# Autodesk Inventor assembly: Project Integration copy
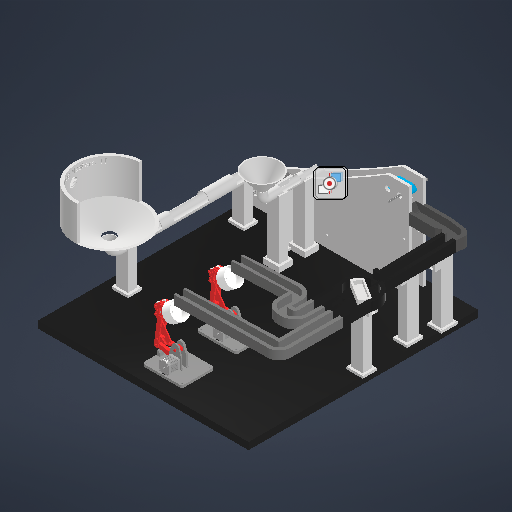
[picture p0: Inventor's stored thumbnail of the model, 512x512]
Saved by Autodesk Inventor 2025.2 (Build 292293000, 293)
## iProperties
Created: 2026-04-17
Part Number: Project Integration copy
Document SubType Name: Assembly
Designer: manon
Author: manon
## Documents named in this file (19)
- C:\Users\osama\Downloads\Project Integration copy .iam
- C:\Users\osama\Downloads\base.ipt
- C:\Users\osama\Downloads\Sorting Path.ipt
- C:\Users\osama\Downloads\Sorting Gate Edited (1).ipt
- C:\Users\osama\Downloads\Assembly Micro Servo MG90S (2) (1).iam
- C:\Users\osama\Downloads\SG90 Horn.ipt
- C:\Users\osama\Downloads\lifting assembly.iam
- C:\Users\osama\Downloads\Path to Sorting Final.ipt
- C:\Users\osama\Downloads\Left Path Final.ipt
- C:\Users\osama\Downloads\Right Path Final.ipt
- C:\Users\osama\Downloads\select support through rabie.ipt
- C:\Users\osama\Downloads\hoop.ipt
- C:\Users\osama\Downloads\support of collector.ipt
- C:\Users\osama\Downloads\path to lifting.ipt
- C:\Users\osama\Downloads\mg996R_v2.ipt
- C:\Users\osama\Downloads\starting point.ipt
- C:\Users\osama\Downloads\Full Assembly.ipt
- C:\Users\osama\Downloads\support of collector copy.ipt
- C:\Users\osama\Downloads\scoop.ipt
## Components (25 placed, 18 different names)
1. base:2 — Mate:26, Mate:27, Mate:57, Mate:58, Mate:62, Mate:68, Mate:72, Mate:76, Mate:88, Mate:89, Mate:96, Mate:99, Mate:100, Mate:101
2. Sorting Path:1 — Mate:5, Mate:6, Mate:43, Mate:44, Mate:45, Mate:46, Mate:47, Mate:48, Mate:50, Mate:55, Mate:90, Mate:91
3. Sorting Gate Edited (1):1 — Mate:5, Mate:6, Rigid:1
4. Assembly Micro Servo MG90S (2) (1):1 [sub-assembly] — Mate:7, Mate:8
5. SG90 Horn:2 — Mate:7, Mate:8, Rigid:1
6. lifting assembly:1 [sub-assembly] — Mate:26, Mate:27, Mate:28, Mate:29, Mate:31
7. Path to Sorting Final:1 — Mate:28, Mate:29, Mate:31
8. Left Path Final:1 — Mate:46, Mate:47, Mate:48
9. Right Path Final:1 — Mate:43, Mate:44, Mate:45
10. select support through rabie:1 — Mate:50, Mate:90
11. select support through rabie:2 — Mate:89, Mate:91
12. select support through rabie:3 — Mate:55, Mate:88
13. hoop:1
14. support of collector:1 — Mate:58, Mate:62
15. support of collector:2 — Mate:57
16. path to lifting:1
17. mg996R_v2:1 — Mate:73, Mate:74, Mate:75, Mate:77, Mate:78, Mate:87
18. starting point:1 — Mate:79, Mate:85
19. Full Assembly:1 — Mate:68, Mate:76, Mate:92, Mate:96, Mate:97
20. Full Assembly:2 — Mate:93, Mate:94, Mate:95
21. select support through rabie:4 — Mate:72, Mate:73, Mate:74, Mate:75, Mate:77, Mate:78, Mate:87
22. support of collector copy:1 — Mate:79, Mate:99, Mate:100
23. support of collector copy:2 — Mate:85, Mate:101
24. scoop:1 — Mate:92, Mate:97
25. scoop:2 — Mate:93, Mate:94, Mate:95
## Relationships (45: Mate 44, WeldJoint 1)
- Mate:5: Sorting Path:1 ↔ Sorting Gate Edited (1):1
- Mate:6: Sorting Path:1 ↔ Sorting Gate Edited (1):1
- Mate:7: Assembly Micro Servo MG90S (2) (1):1 ↔ SG90 Horn:2
- Mate:8: Assembly Micro Servo MG90S (2) (1):1 ↔ SG90 Horn:2
- Rigid:1 [WeldJoint]: Sorting Gate Edited (1):1 ↔ SG90 Horn:2
- Mate:26 (22 mm): base:2 ↔ lifting assembly:1
- Mate:27: base:2 ↔ lifting assembly:1
- Mate:28: lifting assembly:1 ↔ Path to Sorting Final:1
- Mate:29: lifting assembly:1 ↔ Path to Sorting Final:1
- Mate:31: lifting assembly:1 ↔ Path to Sorting Final:1
- Mate:43: Sorting Path:1 ↔ Right Path Final:1
- Mate:44: Sorting Path:1 ↔ Right Path Final:1
- Mate:45: Sorting Path:1 ↔ Right Path Final:1
- Mate:46: Sorting Path:1 ↔ Left Path Final:1
- Mate:47: Sorting Path:1 ↔ Left Path Final:1
- Mate:48: Sorting Path:1 ↔ Left Path Final:1
- Mate:50: Sorting Path:1 ↔ select support through rabie:1
- Mate:55: Sorting Path:1 ↔ select support through rabie:3
- Mate:57: base:2 ↔ support of collector:2
- Mate:58: base:2 ↔ support of collector:1
- Mate:62 (40 mm): base:2 ↔ support of collector:1
- Mate:68: base:2 ↔ Full Assembly:1
- Mate:72: base:2 ↔ select support through rabie:4
- Mate:73: mg996R_v2:1 ↔ select support through rabie:4
- Mate:74: mg996R_v2:1 ↔ select support through rabie:4
- Mate:75: mg996R_v2:1 ↔ select support through rabie:4
- Mate:76 (55 mm): base:2 ↔ Full Assembly:1
- Mate:77: mg996R_v2:1 ↔ select support through rabie:4
- Mate:78 (10.6 mm): mg996R_v2:1 ↔ select support through rabie:4
- Mate:79: starting point:1 ↔ support of collector copy:1
- Mate:85: starting point:1 ↔ support of collector copy:2
- Mate:87: mg996R_v2:1 ↔ select support through rabie:4
- Mate:88: base:2 ↔ select support through rabie:3
- Mate:89: base:2 ↔ select support through rabie:2
- Mate:90: Sorting Path:1 ↔ select support through rabie:1
- Mate:91: Sorting Path:1 ↔ select support through rabie:2
- Mate:92: Full Assembly:1 ↔ scoop:1
- Mate:93: Full Assembly:2 ↔ scoop:2
- Mate:94 (5 mm): Full Assembly:2 ↔ scoop:2
- Mate:95: Full Assembly:2 ↔ scoop:2
- Mate:96 (560 mm): base:2 ↔ Full Assembly:1
- Mate:97: Full Assembly:1 ↔ scoop:1
- Mate:99 (270 mm): base:2 ↔ support of collector copy:1
- Mate:100: base:2 ↔ support of collector copy:1
- Mate:101: base:2 ↔ support of collector copy:2
